# Autodesk Inventor assembly: ObudowaNowa
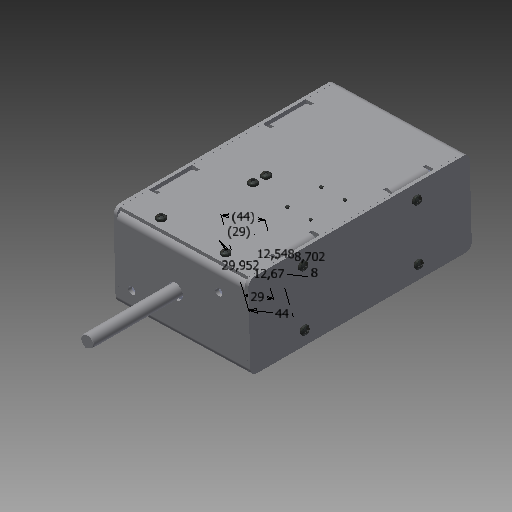
[picture p0: Inventor's stored thumbnail of the model, 512x512]
Saved by Autodesk Inventor 2019.4 (Build 234330000, 330)
## iProperties
Created: 2020-08-21
Part Number: ObudowaNowa
Material: Ogólny
Document SubType Name: Assembly
Designer: barto
Author: barto
## Documents named in this file (24)
- F:\GitHub\MUMv2\Equatorial-Mount-MUM\Mechanika\Moduł obrotu DEK Bartek\odBartka\ObudowaNowa.iam
- F:\GitHub\MUMv2\Equatorial-Mount-MUM\Mechanika\Moduł obrotu DEK Bartek\odBartka\GlownaObudowa.ipt
- F:\GitHub\MUMv2\Equatorial-Mount-MUM\Mechanika\Moduł obrotu DEK Bartek\odBartka\UCFL-201.ipt
- F:\GitHub\MUMv2\Equatorial-Mount-MUM\Mechanika\Moduł obrotu DEK Bartek\odBartka\ModulSilnika.iam
- F:\GitHub\MUMv2\Equatorial-Mount-MUM\Mechanika\Moduł obrotu DEK Bartek\odBartka\ModulWalkaNapinajacego.iam
- F:\GitHub\MUMv2\Equatorial-Mount-MUM\Mechanika\Moduł obrotu DEK Bartek\odBartka\pasekturbonowy.iam
- F:\GitHub\MUMv2\Equatorial-Mount-MUM\Mechanika\Moduł obrotu DEK Bartek\odBartka\ModulDuzegoKola.iam
- F:\GitHub\MUMv2\Equatorial-Mount-MUM\Mechanika\Moduł obrotu DEK Bartek\odBartka\DIN 471 - 12 x 1(1).ipt
- F:\GitHub\MUMv2\Equatorial-Mount-MUM\Mechanika\Moduł obrotu DEK Bartek\odBartka\uchwytDoNapinacza.ipt
- F:\GitHub\MUMv2\Equatorial-Mount-MUM\Mechanika\Moduł obrotu DEK Bartek\odBartka\Połączenie gwintowe1.iam
- F:\GitHub\MUMv2\Equatorial-Mount-MUM\Mechanika\Moduł obrotu DEK Bartek\odBartka\Połączenie gwintowe2.iam
- F:\GitHub\MUMv2\Equatorial-Mount-MUM\Mechanika\Moduł obrotu DEK Bartek\odBartka\Połączenie gwintowe3.iam
- F:\GitHub\MUMv2\Equatorial-Mount-MUM\Mechanika\Moduł obrotu DEK Bartek\odBartka\Połączenie gwintowe4.iam
- F:\GitHub\MUMv2\Equatorial-Mount-MUM\Mechanika\Moduł obrotu DEK Bartek\odBartka\Połączenie gwintowe5.iam
- F:\GitHub\MUMv2\Equatorial-Mount-MUM\Mechanika\Moduł obrotu DEK Bartek\odBartka\Połączenie gwintowe6.iam
- F:\GitHub\MUMv2\Equatorial-Mount-MUM\Mechanika\Moduł obrotu DEK Bartek\odBartka\Połączenie gwintowe7.iam
- F:\GitHub\MUMv2\Equatorial-Mount-MUM\Mechanika\Moduł obrotu DEK Bartek\odBartka\Połączenie gwintowe8.iam
- F:\GitHub\MUMv2\Equatorial-Mount-MUM\Mechanika\Moduł obrotu DEK Bartek\odBartka\Połączenie gwintowe9.iam
- F:\GitHub\MUMv2\Equatorial-Mount-MUM\Mechanika\Moduł obrotu DEK Bartek\odBartka\Połączenie gwintowe10.iam
- F:\GitHub\MUMv2\Equatorial-Mount-MUM\Mechanika\Moduł obrotu DEK Bartek\odBartka\ZaslepkaObudowa.ipt
- F:\GitHub\MUMv2\Equatorial-Mount-MUM\Mechanika\Moduł obrotu DEK Bartek\odBartka\Połączenie gwintowe11.iam
- F:\GitHub\MUMv2\Equatorial-Mount-MUM\Mechanika\Moduł obrotu DEK Bartek\odBartka\Połączenie gwintowe12.iam
- F:\GitHub\MUMv2\Equatorial-Mount-MUM\Mechanika\Moduł obrotu DEK Bartek\odBartka\Połączenie gwintowe13.iam
- F:\GitHub\MUMv2\Equatorial-Mount-MUM\Mechanika\Moduł obrotu DEK Bartek\odBartka\Połączenie gwintowe14.iam
## Components (30 placed, 10 different names)
1. GlownaObudowa:1 — Zestawiające:9, Zestawiające:13, Zestawiające:16, Zestawiające:24, Zestawiające:25, Zestawiające:26, Zestawiające:27, Zestawiające:28, Zestawiające:29, Zestawiające:32, Zestawiające:40, Zestawiające:42, Zestawiające:43, Zestawiające:44, Zestawiające:45, Zestawiające:46, Zestawiające:47, Zestawiające:49, Zestawiające:51, Zestawiające:53, Zestawiające:55, Zestawiające:56, Zestawiające:57, Mate:66, Mate:67, Mate:68, Mate:69
2. ModulSilnika:1 [sub-assembly] — Zestawiające:13, Równoległe:1, Zestawiające:12, Zestawiające:16, Zestawiające:48, Zestawiające:50, Zestawiające:52, Zestawiające:54
3. ModulWalkaNapinajacego:1 [sub-assembly] — Zestawiające:15, Zestawiające:33, Zestawiające:34, Zestawiające:35, Styczny:1, Zestawiające:36, Zestawiające:38, Zestawiające:39
4. pasekturbonowy:1 [sub-assembly] — Zestawiające:10, Zestawiające:11, Zestawiające:12, Zestawiające:15, Styczny:1
5. ModulDuzegoKola:1 [sub-assembly] — Równoległe:1, Zestawiające:9, Zestawiające:10, Zestawiające:11, Zestawiające:23, Zestawiające:30
6. DIN 471 > 9mm <= 300mm 12 x 1:1 — Zestawiające:23
7. UCFL-201:1 — Zestawiające:24, Zestawiające:25, Zestawiające:26
8. UCFL-201:2 — Zestawiające:27, Zestawiające:28, Zestawiające:29, Zestawiające:31
9. DIN 471 > 9mm <= 300mm 12 x 1:2 — Zestawiające:30, Zestawiające:31
10. uchwytDoNapinacza:1 — Zestawiające:32, Zestawiające:33, Zestawiające:34, Zestawiające:35, Zestawiające:37, Zestawiające:41
11. Połączenie gwintowe:1 [sub-assembly] — Zestawiające:36, Zestawiające:37
12. Połączenie gwintowe:2 [sub-assembly] — Zestawiające:38, Zestawiające:39
13. Połączenie gwintowe:3 [sub-assembly] — Zestawiające:40, Zestawiające:41
14. Połączenie gwintowe:4 [sub-assembly] — Zestawiające:42, Zestawiające:43
15. Połączenie gwintowe:5 [sub-assembly] — Zestawiające:44, Zestawiające:45
16. Połączenie gwintowe:6 [sub-assembly] — Zestawiające:46, Zestawiające:47
17. Połączenie gwintowe:7 [sub-assembly] — Zestawiające:48, Zestawiające:49
18. Połączenie gwintowe:8 [sub-assembly] — Zestawiające:50, Zestawiające:51
19. Połączenie gwintowe:9 [sub-assembly] — Zestawiające:52, Zestawiające:53
20. Połączenie gwintowe:10 [sub-assembly] — Zestawiające:54, Zestawiające:55
21. ZaslepkaObudowa:1 — Zestawiające:56, Zestawiające:57, Zestawiające:58, Zestawiające:59, Zestawiające:60, Zestawiające:61, Zestawiające:62, Zestawiające:63, Zestawiające:64, Zestawiające:65
22. Połączenie gwintowe:11 [sub-assembly] — Zestawiające:58, Zestawiające:59
23. Połączenie gwintowe:12 [sub-assembly] — Zestawiające:60, Zestawiające:61, Mate:69
24. Połączenie gwintowe:13 [sub-assembly] — Zestawiające:62, Zestawiające:63
25. Połączenie gwintowe:14 [sub-assembly] — Zestawiające:64, Zestawiające:65
26. ZaslepkaObudowa:2 — Mate:66, Mate:67, Mate:68, Mate:70, Mate:71, Mate:72, Mate:73, Mate:74, Mate:75, Mate:76, Mate:77
27. Połączenie gwintowe:15 [sub-assembly] — Mate:72, Mate:75
28. Połączenie gwintowe:16 [sub-assembly] — Mate:73, Mate:76
29. Połączenie gwintowe:17 [sub-assembly] — Mate:70, Mate:77
30. Połączenie gwintowe:18 [sub-assembly] — Mate:71, Mate:74
## Relationships (64: Mate 62, Flush 1, Tangent 1)
- Zestawiające:13 [Mate]: GlownaObudowa:1 ↔ ModulSilnika:1
- Równoległe:1 [Flush]: ModulSilnika:1 ↔ ModulDuzegoKola:1
- Zestawiające:9 [Mate]: GlownaObudowa:1 ↔ ModulDuzegoKola:1
- Zestawiające:10 [Mate] (0.5 mm): pasekturbonowy:1 ↔ ModulDuzegoKola:1
- Zestawiające:11 [Mate]: pasekturbonowy:1 ↔ ModulDuzegoKola:1
- Zestawiające:12 [Mate]: ModulSilnika:1 ↔ pasekturbonowy:1
- Zestawiające:15 [Mate] (0.5 mm): ModulWalkaNapinajacego:1 ↔ pasekturbonowy:1
- Zestawiające:16 [Mate] (60 mm): GlownaObudowa:1 ↔ ModulSilnika:1
- Zestawiające:23 [Mate]: ModulDuzegoKola:1 ↔ DIN 471 > 9mm <= 300mm 12 x 1:1
- Zestawiające:24 [Mate]: GlownaObudowa:1 ↔ UCFL-201:1
- Zestawiające:25 [Mate]: GlownaObudowa:1 ↔ UCFL-201:1
- Zestawiające:26 [Mate]: GlownaObudowa:1 ↔ UCFL-201:1
- Zestawiające:27 [Mate]: GlownaObudowa:1 ↔ UCFL-201:2
- Zestawiające:28 [Mate]: GlownaObudowa:1 ↔ UCFL-201:2
- Zestawiające:29 [Mate]: GlownaObudowa:1 ↔ UCFL-201:2
- Zestawiające:30 [Mate]: ModulDuzegoKola:1 ↔ DIN 471 > 9mm <= 300mm 12 x 1:2
- Zestawiające:31 [Mate]: UCFL-201:2 ↔ DIN 471 > 9mm <= 300mm 12 x 1:2
- Zestawiające:32 [Mate]: GlownaObudowa:1 ↔ uchwytDoNapinacza:1
- Zestawiające:33 [Mate]: ModulWalkaNapinajacego:1 ↔ uchwytDoNapinacza:1
- Zestawiające:34 [Mate]: ModulWalkaNapinajacego:1 ↔ uchwytDoNapinacza:1
- Zestawiające:35 [Mate]: ModulWalkaNapinajacego:1 ↔ uchwytDoNapinacza:1
- Styczny:1 [Tangent]: ModulWalkaNapinajacego:1 ↔ pasekturbonowy:1
- Zestawiające:36 [Mate]: ModulWalkaNapinajacego:1 ↔ Połączenie gwintowe:1
- Zestawiające:37 [Mate]: uchwytDoNapinacza:1 ↔ Połączenie gwintowe:1
- Zestawiające:38 [Mate]: ModulWalkaNapinajacego:1 ↔ Połączenie gwintowe:2
- Zestawiające:39 [Mate]: ModulWalkaNapinajacego:1 ↔ Połączenie gwintowe:2
- Zestawiające:40 [Mate]: GlownaObudowa:1 ↔ Połączenie gwintowe:3
- Zestawiające:41 [Mate]: uchwytDoNapinacza:1 ↔ Połączenie gwintowe:3
- Zestawiające:42 [Mate]: GlownaObudowa:1 ↔ Połączenie gwintowe:4
- Zestawiające:43 [Mate]: GlownaObudowa:1 ↔ Połączenie gwintowe:4
- Zestawiające:44 [Mate]: GlownaObudowa:1 ↔ Połączenie gwintowe:5
- Zestawiające:45 [Mate]: GlownaObudowa:1 ↔ Połączenie gwintowe:5
- Zestawiające:46 [Mate]: GlownaObudowa:1 ↔ Połączenie gwintowe:6
- Zestawiające:47 [Mate]: GlownaObudowa:1 ↔ Połączenie gwintowe:6
- Zestawiające:48 [Mate]: ModulSilnika:1 ↔ Połączenie gwintowe:7
- Zestawiające:49 [Mate]: GlownaObudowa:1 ↔ Połączenie gwintowe:7
- Zestawiające:50 [Mate]: ModulSilnika:1 ↔ Połączenie gwintowe:8
- Zestawiające:51 [Mate]: GlownaObudowa:1 ↔ Połączenie gwintowe:8
- Zestawiające:52 [Mate]: ModulSilnika:1 ↔ Połączenie gwintowe:9
- Zestawiające:53 [Mate]: GlownaObudowa:1 ↔ Połączenie gwintowe:9
- Zestawiające:54 [Mate]: ModulSilnika:1 ↔ Połączenie gwintowe:10
- Zestawiające:55 [Mate]: GlownaObudowa:1 ↔ Połączenie gwintowe:10
- Zestawiające:56 [Mate]: GlownaObudowa:1 ↔ ZaslepkaObudowa:1
- Zestawiające:57 [Mate]: GlownaObudowa:1 ↔ ZaslepkaObudowa:1
- Zestawiające:58 [Mate]: ZaslepkaObudowa:1 ↔ Połączenie gwintowe:11
- Zestawiające:59 [Mate]: ZaslepkaObudowa:1 ↔ Połączenie gwintowe:11
- Zestawiające:60 [Mate]: ZaslepkaObudowa:1 ↔ Połączenie gwintowe:12
- Zestawiające:61 [Mate]: ZaslepkaObudowa:1 ↔ Połączenie gwintowe:12
- Zestawiające:62 [Mate]: ZaslepkaObudowa:1 ↔ Połączenie gwintowe:13
- Zestawiające:63 [Mate]: ZaslepkaObudowa:1 ↔ Połączenie gwintowe:13
- Zestawiające:64 [Mate]: ZaslepkaObudowa:1 ↔ Połączenie gwintowe:14
- Zestawiające:65 [Mate]: ZaslepkaObudowa:1 ↔ Połączenie gwintowe:14
- Mate:66: GlownaObudowa:1 ↔ ZaslepkaObudowa:2
- Mate:67: GlownaObudowa:1 ↔ ZaslepkaObudowa:2
- Mate:68: GlownaObudowa:1 ↔ ZaslepkaObudowa:2
- Mate:69: GlownaObudowa:1 ↔ Połączenie gwintowe:12
- Mate:70: ZaslepkaObudowa:2 ↔ Połączenie gwintowe:17
- Mate:71: ZaslepkaObudowa:2 ↔ Połączenie gwintowe:18
- Mate:72: ZaslepkaObudowa:2 ↔ Połączenie gwintowe:15
- Mate:73: ZaslepkaObudowa:2 ↔ Połączenie gwintowe:16
- Mate:74: ZaslepkaObudowa:2 ↔ Połączenie gwintowe:18
- Mate:75: ZaslepkaObudowa:2 ↔ Połączenie gwintowe:15
- Mate:76: ZaslepkaObudowa:2 ↔ Połączenie gwintowe:16
- Mate:77: ZaslepkaObudowa:2 ↔ Połączenie gwintowe:17
